# Autodesk Inventor assembly: EnsambleTuberiaCalderin
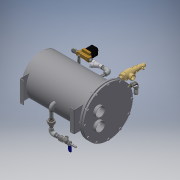
[picture p0: Inventor's stored thumbnail of the model, 180x180]
Saved by Autodesk Inventor 2017 (Build 210142000, 142)
## iProperties
Created: 2021-06-28
Part Number: EnsambleTuberiaCalderin
Document SubType Name: Assembly
Designer: USUARIO
Author: USUARIO
## Documents named in this file (19)
- D:\Laboratorio\Autoclave\Autoclave Horizontal\Con Precamara\2021\Autoclave 110L Biocacol OP2021110 #0045886XX\Modelo\Planos\EnsambleTuberiaCalderin.iam
- D:\Laboratorio\Autoclave\Autoclave Horizontal\Con Precamara\2021\Autoclave 110L Biocacol OP2021110 #0045886XX\Modelo\ENSAMBLE CALDERIN ACH-110L-2021-P.iam
- C:\Modelos 3D y DXF\Racores\B122 1-2x1-2.ipt
- C:\Modelos 3D y DXF\Danfoss EV210B\DANFOS EV225B.ipt
- C:\Modelos 3D y DXF\Filtro en Y\Filtro Y 1-2'' Inox.ipt
- C:\Modelos 3D y DXF\Racores\Niple 1-2x3.ipt
- C:\Modelos 3D y DXF\Racores\User Library-codo a 90 de 1-2-Rosc.ipt
- C:\Modelos 3D y DXF\Racores\B69 1-4x1-4.iam
- C:\Modelos 3D y DXF\Racores\T 0.25.ipt
- C:\Modelos 3D y DXF\Racores\union macho macho 0.25.ipt
- C:\Modelos 3D y DXF\Racores\1-2-1-2-SwagelokCompany-3D-06-16-2021.ipt
- C:\Modelos 3D y DXF\Racores\User Library-Tee_Class300.ipt
- C:\Modelos 3D y DXF\Racores\TRAMPA SPIRAX SARCO.ipt
- C:\Modelos 3D y DXF\Racores\B3 1-2x1-2.ipt
- C:\Modelos 3D y DXF\Racores\User Library-Valvula-segur-popup-1-2.ipt
- C:\Modelos 3D y DXF\Racores\Check Valve 0.5.ipt
- C:\Modelos 3D y DXF\Racores\CodoCalle.iam
- C:\Modelos 3D y DXF\Racores\Universal1-2.ipt
- C:\Modelos 3D y DXF\Racores\User Library-Valve-1.ipt
## Components (34 placed, 18 different names)
1. ENSAMBLE CALDERIN ACH-110L-2021-P:1 [sub-assembly]
2. B122 1-2x1-2:1
3. DANFOS EV225B:1
4. Filtro Y 1-2'' Inox:1
5. B122 1-2x1-2:2
6. Niple 1-2x3:1
7. User Library-codo a 90 de 1-2-Rosc:1
8. B69 1-4x1-4:1 [sub-assembly]
9. T 0.25:1
10. union macho macho 0.25:1
11. B69 1-4x1-4:2 [sub-assembly]
12. B69 1-4x1-4:3 [sub-assembly]
13. 1-2-1-2-SwagelokCompany-3D-06-16-2021:1
14. B122 1-2x1-2:3
15. User Library-Tee_Class300:1
16. B122 1-2x1-2:4
17. Filtro Y 1-2'' Inox:2
18. TRAMPA SPIRAX SARCO:1
19. B3 1-2x1-2:1
20. User Library-Valvula-segur-popup-1-2:1
21. B122 1-2x1-2:5
22. Check Valve 0.5:1
23. 1-2-1-2-SwagelokCompany-3D-06-16-2021:2
24. CodoCalle:1 [sub-assembly]
25. Niple 1-2x3:2
26. Universal1-2:1
27. B122 1-2x1-2:6
28. User Library-codo a 90 de 1-2-Rosc:2
29. User Library-Valve-1:1
30. B122 1-2x1-2:7
31. B3 1-2x1-2:2
32. B69 1-4x1-4:4 [sub-assembly]
33. B69 1-4x1-4:5 [sub-assembly]
34. B69 1-4x1-4:6 [sub-assembly]
## Relationships (33: Insert 33)
- [Insert] (-9 mm): B122 1-2x1-2:1 ↔ DANFOS EV225B:1
- [Insert] (7 mm): Filtro Y 1-2'' Inox:1 ↔ B122 1-2x1-2:2
- [Insert] (-7 mm): B122 1-2x1-2:1 ↔ Filtro Y 1-2'' Inox:1
- [Insert] (-9 mm): ENSAMBLE CALDERIN ACH-110L-2021-P:1 ↔ Niple 1-2x3:1
- [Insert] (-10 mm): Niple 1-2x3:1 ↔ User Library-codo a 90 de 1-2-Rosc:1
- [Insert] (-12 mm): B122 1-2x1-2:2 ↔ User Library-codo a 90 de 1-2-Rosc:1
- [Insert] (-9 mm): ENSAMBLE CALDERIN ACH-110L-2021-P:1 ↔ B69 1-4x1-4:1
- [Insert] (-7 mm): ENSAMBLE CALDERIN ACH-110L-2021-P:1 ↔ union macho macho 0.25:1
- [Insert] (-7 mm): T 0.25:1 ↔ union macho macho 0.25:1
- [Insert] (-7 mm): T 0.25:1 ↔ B69 1-4x1-4:3
- [Insert] (-7 mm): T 0.25:1 ↔ B69 1-4x1-4:2
- [Insert] (9 mm): DANFOS EV225B:1 ↔ 1-2-1-2-SwagelokCompany-3D-06-16-2021:1
- [Insert] (12 mm): B122 1-2x1-2:3 ↔ User Library-Tee_Class300:1
- [Insert] (-9 mm): User Library-Tee_Class300:1 ↔ B122 1-2x1-2:4
- [Insert] (-9 mm): ENSAMBLE CALDERIN ACH-110L-2021-P:1 ↔ B122 1-2x1-2:4
- [Insert] (-9 mm): Filtro Y 1-2'' Inox:2 ↔ TRAMPA SPIRAX SARCO:1
- [Insert] (-7 mm): B122 1-2x1-2:3 ↔ Filtro Y 1-2'' Inox:2
- [Insert] (-7 mm): TRAMPA SPIRAX SARCO:1 ↔ B3 1-2x1-2:1
- [Insert] (-9 mm): User Library-Tee_Class300:1 ↔ User Library-Valvula-segur-popup-1-2:1
- [Insert] (-7 mm): B122 1-2x1-2:5 ↔ Check Valve 0.5:1
- [Insert] (-9 mm): ENSAMBLE CALDERIN ACH-110L-2021-P:1 ↔ B122 1-2x1-2:5
- [Insert] (9 mm): 1-2-1-2-SwagelokCompany-3D-06-16-2021:2 ↔ CodoCalle:1
- [Insert] (-7 mm): Check Valve 0.5:1 ↔ CodoCalle:1
- [Insert] (-12 mm): Niple 1-2x3:2 ↔ Universal1-2:1
- [Insert] (-12 mm): ENSAMBLE CALDERIN ACH-110L-2021-P:1 ↔ Niple 1-2x3:2
- [Insert] (-12 mm): B122 1-2x1-2:6 ↔ User Library-codo a 90 de 1-2-Rosc:2
- [Insert] (-12 mm): Universal1-2:1 ↔ B122 1-2x1-2:6
- [Insert] (-7 mm): User Library-Valve-1:1 ↔ B122 1-2x1-2:7
- [Insert] (-7 mm): User Library-Valve-1:1 ↔ B3 1-2x1-2:2
- [Insert] (-7 mm): User Library-codo a 90 de 1-2-Rosc:2 ↔ B122 1-2x1-2:7
- [Insert] (-7 mm): ENSAMBLE CALDERIN ACH-110L-2021-P:1 ↔ B69 1-4x1-4:4
- [Insert] (-7 mm): ENSAMBLE CALDERIN ACH-110L-2021-P:1 ↔ B69 1-4x1-4:5
- [Insert] (-7 mm): ENSAMBLE CALDERIN ACH-110L-2021-P:1 ↔ B69 1-4x1-4:6
## Named parameters: d173_d159 = -12 mm, d175_d124 = -7 mm, d176_d126 = -7 mm, d81_d38_d9 = -9 mm, d82_d26_d12 = 7 mm, d113_d31 = -9 mm, d114_d28_d3 = 12 mm, d116_d59 = -9 mm, d120_d54_d7 = -7 mm, d122_d101 = 9 mm
